# Autodesk Inventor assembly: CLAW
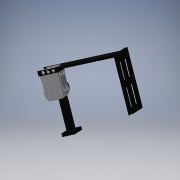
[picture p0: Inventor's stored thumbnail of the model, 180x180]
Saved by Autodesk Inventor 2016 (Build 200138000, 138)
## iProperties
Created: 2016-03-31
Part Number: CLAW
Document SubType Name: Assembly
Designer: mkepler
Author: mkepler
## Documents named in this file (5)
- C:\Users\mkepler\Google Drive\Michael Kepler\College\ECE\ECE 590\Project 2\Inventor Files\Claw\CLAW.iam
- C:\Users\mkepler\Google Drive\Michael Kepler\College\ECE\ECE 590\Project 2\Inventor Files\Claw\GrapperRight.ipt
- C:\Users\mkepler\Google Drive\Michael Kepler\College\ECE\ECE 590\Project 2\Inventor Files\xl320Servo.ipt
- C:\Users\mkepler\Google Drive\Michael Kepler\College\ECE\ECE 590\Project 2\Inventor Files\Claw\GripperLeftContact.ipt
- C:\Users\mkepler\Google Drive\Michael Kepler\College\ECE\ECE 590\Project 2\Inventor Files\Claw\GripperLeft.ipt
## Components (4 placed, 4 different names)
1. GrapperRight:1 — Insert:1, Insert:2
2. xl320Servo:1 — Insert:1, Insert:2, Insert:3, Mate:5
3. GripperLeftContact:1 — Mate:3, Mate:4, Mate:6
4. GripperLeft:1 — Mate:3, Mate:4, Insert:3, Mate:5, Mate:6
## Relationships (7: Mate 4, Insert 3)
- Insert:1: GrapperRight:1 ↔ xl320Servo:1
- Insert:2: GrapperRight:1 ↔ xl320Servo:1
- Mate:3: GripperLeftContact:1 ↔ GripperLeft:1
- Mate:4: GripperLeftContact:1 ↔ GripperLeft:1
- Insert:3: xl320Servo:1 ↔ GripperLeft:1
- Mate:5: xl320Servo:1 ↔ GripperLeft:1
- Mate:6: GripperLeftContact:1 ↔ GripperLeft:1
